# Autodesk Inventor assembly: Z_GANTRY
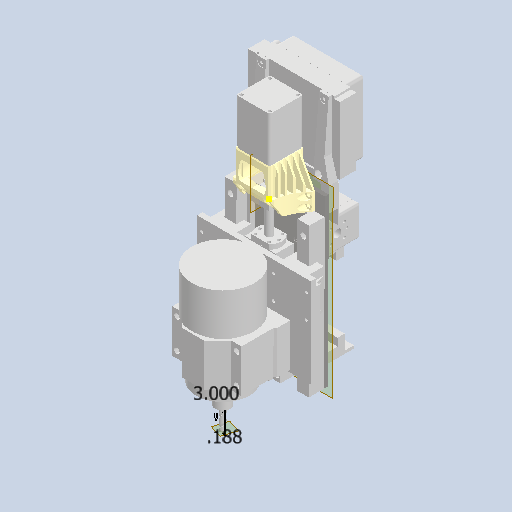
[picture p0: Inventor's stored thumbnail of the model, 512x512]
Saved by Autodesk Inventor 2023 (Build 270158000, 158)
## iProperties
Created: 2023-06-21
Part Number: Z_GANTRY
Document SubType Name: Assembly
Designer: plebbb
Author: plebbb
## Documents named in this file (17)
- G:\CNC PROJECT\CNC_Project\Z_GANTRY.iam
- G:\CNC PROJECT\CNC_Project\Ballscrew_Assembly_1204.iam
- G:\CNC PROJECT\CNC_Project\2x3_L_Bracket.ipt
- G:\CNC PROJECT\CNC_Project\HGW20CC_Slider.ipt
- G:\CNC PROJECT\CNC_Project\HGW20CC_Rail_300mm.ipt
- G:\CNC PROJECT\CNC_Project\Z_PLATE.iam
- G:\CNC PROJECT\CNC_Project\SFU1204-300.ipt
- G:\CNC PROJECT\CNC_Project\Spindle.ipt
- G:\CNC PROJECT\CNC_Project\BK10.ipt
- G:\CNC PROJECT\CNC_Project\Drill_Bit.ipt
- G:\CNC PROJECT\CNC_Project\Z_Gantry_Plate_Spaced.iam
- G:\CNC PROJECT\CNC_Project\SFU1204_Nut.ipt
- G:\CNC PROJECT\CNC_Project\DSG12H.ipt
- G:\CNC PROJECT\CNC_Project\BF10.ipt
- G:\CNC PROJECT\CNC_Project\Z_Motor_Holder.ipt
- G:\CNC PROJECT\CNC_Project\Nema23_Short.ipt
- G:\CNC PROJECT\CNC_Project\Watercooling_System.iam
## Components (17 placed, 16 different names)
1. Ballscrew_Assembly_1204:1 [sub-assembly]
2. 2x3_L_Bracket:1
3. HGW20CC_Slider:1
4. HGW20CC_Rail_300mm:1
5. HGW20CC_Rail_300mm:2
6. Z_PLATE:1 [sub-assembly]
7. SFU1204-300:1
8. Spindle:1
9. BK10:1
10. Drill_Bit:1
11. Z_Gantry_Plate_Spaced:1 [sub-assembly] — Mate:32, Angle:5, Flush:12
12. SFU1204_Nut:1
13. DSG12H:1
14. BF10:1
15. Z_Motor_Holder:1
16. Nema23_Short:1
17. Watercooling_System:1 [sub-assembly] — Mate:32, Angle:5, Flush:12
## Relationships (49: Mate 32, Flush 12, Angle 5)
- [Mate]: 2x3_L_Bracket:1 ↔ HGW20CC_Slider:1
- [Mate]: 2x3_L_Bracket:1 ↔ HGW20CC_Slider:1
- [Mate]: 2x3_L_Bracket:1 ↔ HGW20CC_Slider:1
- [Mate]: Ballscrew_Assembly_1204:1 ↔ Z_Gantry_Plate_Spaced:1
- [Mate]: Ballscrew_Assembly_1204:1 ↔ Z_Gantry_Plate_Spaced:1
- [Mate]: 2x3_L_Bracket:1 ↔ Z_Gantry_Plate_Spaced:1
- [Mate]: Ballscrew_Assembly_1204:1 ↔ Z_Gantry_Plate_Spaced:1
- [Flush]: HGW20CC_Rail_300mm:1 ↔ HGW20CC_Rail_300mm:2
- [Angle] (0 deg): HGW20CC_Rail_300mm:1 ↔ HGW20CC_Rail_300mm:2
- [Angle] (180 deg): HGW20CC_Rail_300mm:1 ↔ Z_Gantry_Plate_Spaced:1
- [Mate]: HGW20CC_Rail_300mm:1 ↔ Z_Gantry_Plate_Spaced:1
- [Mate]: HGW20CC_Rail_300mm:2 ↔ Z_Gantry_Plate_Spaced:1
- [Flush]: HGW20CC_Rail_300mm:1 ↔ Z_Gantry_Plate_Spaced:1
- [Flush]: HGW20CC_Rail_300mm:2 ↔ Z_Gantry_Plate_Spaced:1
- [Flush]: HGW20CC_Rail_300mm:2 ↔ Z_Gantry_Plate_Spaced:1
- [Mate]: HGW20CC_Rail_300mm:2 ↔ Z_PLATE:1
- [Mate]: HGW20CC_Rail_300mm:2 ↔ Z_PLATE:1
- [Flush]: HGW20CC_Rail_300mm:1 ↔ Z_PLATE:1
- [Mate]: SFU1204-300:1 ↔ SFU1204_Nut:1
- [Flush]: SFU1204-300:1 ↔ Z_Gantry_Plate_Spaced:1
- [Mate]: Z_PLATE:1 ↔ Spindle:1
- [Flush] (-20 mm): Z_PLATE:1 ↔ Spindle:1
- [Mate]: SFU1204-300:1 ↔ BK10:1
- [Mate]: Spindle:1 ↔ Drill_Bit:1
- [Mate]: Spindle:1 ↔ Drill_Bit:1
- [Mate] (10 mm): BK10:1 ↔ SFU1204_Nut:1
- [Mate]: SFU1204_Nut:1 ↔ DSG12H:1
- [Mate]: SFU1204_Nut:1 ↔ DSG12H:1
- [Mate]: SFU1204_Nut:1 ↔ DSG12H:1
- [Mate]: Z_PLATE:1 ↔ DSG12H:1
- [Mate]: Z_PLATE:1 ↔ DSG12H:1
- [Mate]: BK10:1 ↔ Z_Gantry_Plate_Spaced:1
- [Flush]: HGW20CC_Rail_300mm:1 ↔ Z_PLATE:1
- [Mate]: Z_Gantry_Plate_Spaced:1 ↔ BF10:1
- [Angle] (0 deg): Z_Gantry_Plate_Spaced:1 ↔ BF10:1
- [Mate]: SFU1204-300:1 ↔ BF10:1
- [Mate]: SFU1204-300:1 ↔ BF10:1
- [Mate]: SFU1204-300:1 ↔ Z_Motor_Holder:1
- [Mate]: Z_Motor_Holder:1 ↔ Nema23_Short:1
- [Mate]: Z_Motor_Holder:1 ↔ Nema23_Short:1
- [Mate]: Z_Motor_Holder:1 ↔ Nema23_Short:1
- [Mate] (2 mm): SFU1204-300:1 ↔ Nema23_Short:1
- [Angle] (0 deg): BK10:1 ↔ Nema23_Short:1
- [Flush] (-22.75 mm): SFU1204-300:1 ↔ BK10:1
- [Flush] (-4 mm): BK10:1 ↔ Z_Gantry_Plate_Spaced:1
- [Flush] (0.15 mm): Z_Gantry_Plate_Spaced:1 ↔ Z_Motor_Holder:1
- Mate:32: Z_Gantry_Plate_Spaced:1 ↔ Watercooling_System:1
- Angle:5 (180 deg): Z_Gantry_Plate_Spaced:1 ↔ Watercooling_System:1
- Flush:12: Z_Gantry_Plate_Spaced:1 ↔ Watercooling_System:1
## Named parameters: d31_d64 = 0 mm, d35_d68 = 0 mm, d36_d69 = 0 mm, d37_d70 = 0 mm, d38_d71 = 0 mm, d39_d72 = 0 mm, d40_d73 = 0 deg, d41_d74 = 180 deg, d42_d79 = 0 mm, d43_d80 = 0 mm, d44_d81 = 0 mm, d45_d83 = 0 mm, d46_d85 = 0 mm, d47_d86 = 0 mm
